# Autodesk Inventor assembly: Assembly1
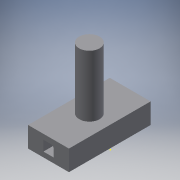
[picture p0: Inventor's stored thumbnail of the model, 180x180]
Saved by Autodesk Inventor 2018.2 (Build 222227000, 227)
## iProperties
Created: 2019-01-20
Part Number: Assembly1
Document SubType Name: Assembly
Designer: faisa
Author: faisa
## Documents named in this file (3)
- C:\Users\faisa\Desktop\Practise\Assembly1.iam
- C:\Users\faisa\Desktop\Practise\Block.ipt
- C:\Users\faisa\Desktop\Practise\peg.ipt
## Components (2 placed, 2 different names)
1. Block:3 — Mate:1, Flush:1
2. peg:1 — Mate:1, Flush:1
## Relationships (2: Mate 1, Flush 1)
- Mate:1: Block:3 ↔ peg:1
- Flush:1: Block:3 ↔ peg:1
